# Autodesk Inventor assembly: Case Top
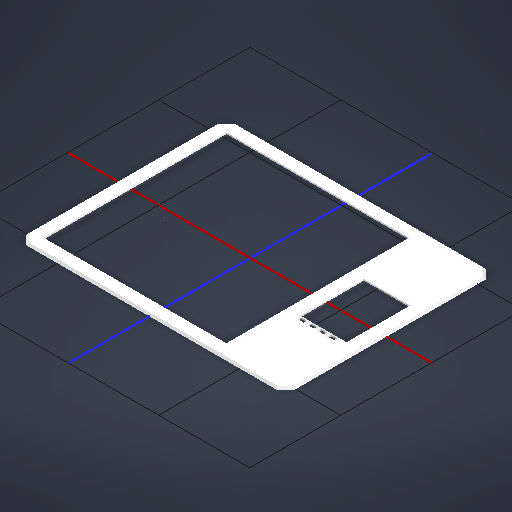
[picture p0: Inventor's stored thumbnail of the model, 512x512]
Saved by Autodesk Inventor 2026 (Build 300175000, 175)
## iProperties
Created: 2025-06-09
Part Number: Case Top
Document SubType Name: Assembly
Designer: ckyiu
Author: ckyiu
## Documents named in this file (5)
- F:\Chessboard-Design\Assemblies\Case\Case Top.iam
- F:\Chessboard-Design\Parts\Case\Top\Case Top BL.ipt
- F:\Chessboard-Design\Parts\Case\Top\Case Top BR.ipt
- F:\Chessboard-Design\Parts\Case\Top\Case Top TL.ipt
- F:\Chessboard-Design\Parts\Case\Top\Case Top TR.ipt
## Components (4 placed, 4 different names)
1. Case Top TL:1 — Mate:1, Flush:1, Flush:2, Mate:2, Flush:3, Flush:4
2. Case Top TR:1 — Mate:1, Flush:1, Flush:2
3. Case Top BL:1 — Mate:2, Flush:3, Flush:4, Mate:3, Flush:5, Flush:6
4. Case Top BR:1 — Mate:3, Flush:5, Flush:6
## Relationships (9: Flush 6, Mate 3)
- Mate:1: Case Top TL:1 ↔ Case Top TR:1
- Flush:1: Case Top TL:1 ↔ Case Top TR:1
- Flush:2: Case Top TL:1 ↔ Case Top TR:1
- Mate:2: Case Top TL:1 ↔ Case Top BL:1
- Flush:3: Case Top TL:1 ↔ Case Top BL:1
- Flush:4: Case Top TL:1 ↔ Case Top BL:1
- Mate:3: Case Top BL:1 ↔ Case Top BR:1
- Flush:5: Case Top BL:1 ↔ Case Top BR:1
- Flush:6: Case Top BL:1 ↔ Case Top BR:1
